# Autodesk Inventor assembly: ArmLoopAssembly
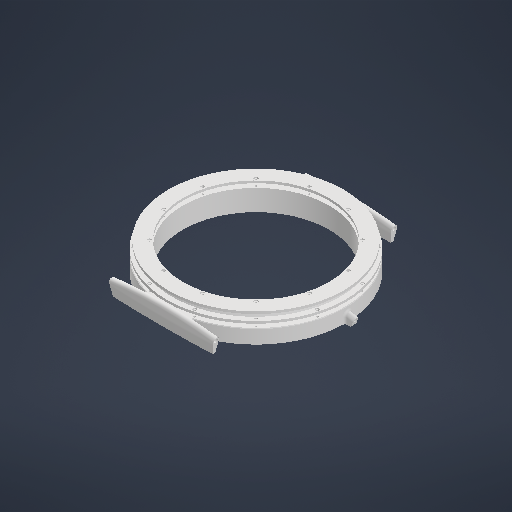
[picture p0: Inventor's stored thumbnail of the model, 512x512]
Saved by Autodesk Inventor 2026.1 (Build 301233020, 233B)
## iProperties
Created: 2025-10-20
Part Number: ArmLoopAssembly
Document SubType Name: Assembly
Designer: skybound
Author: skybound
## Documents named in this file (4)
- C:\Users\skybound\Documents\Projects\Totoro\ArmLoopAssembly.iam
- C:\Users\skybound\Documents\Projects\Totoro\ArmLoopMount.ipt
- C:\Users\skybound\Documents\Projects\Totoro\ArmLoopOuterRing.ipt
- C:\Users\skybound\Documents\Projects\Totoro\ArmLoopInnerRing.ipt
## Components (3 placed, 3 different names)
1. ArmLoopMount:1 — Cylindrical:1, Planar:1, Cylindrical:2, Cylindrical:3, Rotational:1, Cylindrical:4
2. ArmLoopOuterRing:1 — Cylindrical:1, Planar:1, Cylindrical:2
3. ArmLoopInnerRing:1 — Cylindrical:3, Rotational:1, Cylindrical:4
## Relationships (6: CylindricalJoint 4, PlanarJoint 1, RevoluteJoint 1)
- Cylindrical:1: ArmLoopMount:1 ↔ ArmLoopOuterRing:1
- Planar:1 (3 mm): ArmLoopMount:1 ↔ ArmLoopOuterRing:1
- Cylindrical:2: ArmLoopMount:1 ↔ ArmLoopOuterRing:1
- Cylindrical:3: ArmLoopMount:1 ↔ ArmLoopInnerRing:1
- Rotational:1 [RevoluteJoint] (3 mm): ArmLoopMount:1 ↔ ArmLoopInnerRing:1
- Cylindrical:4: ArmLoopMount:1 ↔ ArmLoopInnerRing:1
